# Autodesk Inventor assembly: Ensamblajecaballo abrebottellas1.3
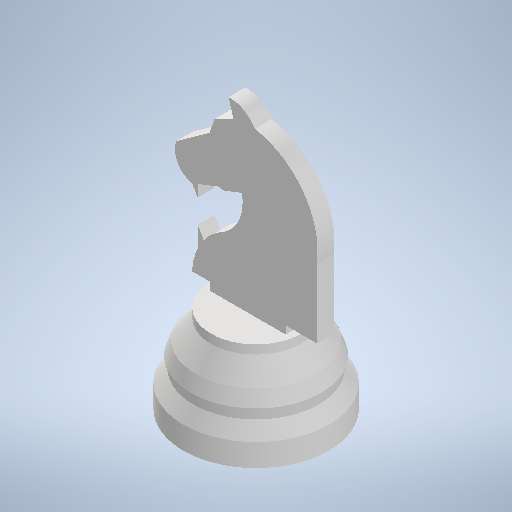
[picture p0: Inventor's stored thumbnail of the model, 512x512]
Saved by Autodesk Inventor 2025.1 (Build 291241000, 241)
## iProperties
Created: 2024-11-01
Part Number: Ensamblajecaballo abrebottellas1.3
Document SubType Name: Assembly
Designer: Octavio
Author: Octavio
## Documents named in this file (3)
- C:\Users\Octavio\Documents\Inventor\CABALLO\Ensambraje Knight 1.3\Ensamblajecaballo abrebottellas1.3.iam
- C:\Users\Octavio\Documents\Inventor\CABALLO\Knght 1.0\KIGTH TOP ABREBOTELLA 1.2.ipt
- C:\Users\Octavio\Documents\Inventor\CABALLO\Knght 1.0\KINGHT BASE 1.1.ipt
## Components (2 placed, 2 different names)
1. KIGTH TOP ABREBOTELLA 1.2:1 — Rígido:1
2. KINGHT BASE 1.1:1 — Rígido:1
## Relationships (1: WeldJoint 1)
- Rígido:1 [WeldJoint] (-1 mm): KIGTH TOP ABREBOTELLA 1.2:1 ↔ KINGHT BASE 1.1:1
